# Autodesk Inventor assembly: FLUGGER R UPSTOP FLAP
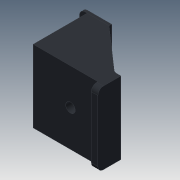
[picture p0: Inventor's stored thumbnail of the model, 180x180]
Saved by Autodesk Inventor 2020.3 (Build 243373000, 373)
## iProperties
RuleStatus: InUse
AfterDocSave0: file://Part Number Cleaner
Created: 2023-03-27
Catalog Web Link: https://www.janelia.org/
Vendor: HHMI: JRC - jET
Document SubType Name: Assembly
Designer: arnoldj
DESIGN DEPARTMENT: HHMI: JRC - jET
ALTERED ITEM PART NUMBER: N/A
ALTERED ITEM VENDOR: N/A
ALTERED ITEM DESCRIPTION: N/A
PART NUMBER - LEGACY: Standard
Author: arnoldj
Revision Number: 0
## Documents named in this file (5)
- C:\_WORKSPACE\DATA\PROJECTS\_PROJECTS BY LAB\CARD (LAB)\FLUGGER\FLUGGER R UPSTOP FLAP.iam
- C:\_WORKSPACE\DATA\PROJECTS\_PROJECTS BY LAB\CARD (LAB)\FLUGGER\FLUGGER TRAY UPSTOP FLAP .ipt
- C:\_WORKSPACE\DATA\COMMON\McMaster\94855A279_LOW-STRENGTH STEEL SQUARE NUT.ipt
- C:\_WORKSPACE\DATA\PROJECTS\_PROJECTS BY LAB\CARD (LAB)\FLUGGER\FL UPSTOP FLAP.ipt
- C:\_WORKSPACE\DATA\COMMON\McMaster\MCMASTER 91771A080 2-56 x437L FHMS SS.ipt
## Components (8 placed, 4 different names)
1. FLUGGER TRAY UPSTOP FLAP :1 — Mate:1, Mate:2, Mate:3, Mate:4, Mate:5, Mate:6, Mate:7, Mate:8, Mate:9
2. 94855A279_LOW-STRENGTH STEEL SQUARE NUT:1 — Mate:1, Mate:4
3. 94855A279_LOW-STRENGTH STEEL SQUARE NUT:2 — Mate:2, Mate:5
4. 94855A279_LOW-STRENGTH STEEL SQUARE NUT:3 — Mate:3, Mate:6
5. FL UPSTOP FLAP:1 — Mate:7, Mate:8, Mate:9, Flush:1, Mate:10, Flush:2, Mate:11, Flush:3, Mate:12
6. MCMASTER 91771A080 2-56 x437L FHMS SS:1 — Flush:3, Mate:12
7. MCMASTER 91771A080 2-56 x437L FHMS SS:2 — Flush:2, Mate:11
8. MCMASTER 91771A080 2-56 x437L FHMS SS:3 — Flush:1, Mate:10
## Relationships (15: Mate 12, Flush 3)
- Mate:1: FLUGGER TRAY UPSTOP FLAP :1 ↔ 94855A279_LOW-STRENGTH STEEL SQUARE NUT:1
- Mate:2: FLUGGER TRAY UPSTOP FLAP :1 ↔ 94855A279_LOW-STRENGTH STEEL SQUARE NUT:2
- Mate:3: FLUGGER TRAY UPSTOP FLAP :1 ↔ 94855A279_LOW-STRENGTH STEEL SQUARE NUT:3
- Mate:4: FLUGGER TRAY UPSTOP FLAP :1 ↔ 94855A279_LOW-STRENGTH STEEL SQUARE NUT:1
- Mate:5: FLUGGER TRAY UPSTOP FLAP :1 ↔ 94855A279_LOW-STRENGTH STEEL SQUARE NUT:2
- Mate:6: FLUGGER TRAY UPSTOP FLAP :1 ↔ 94855A279_LOW-STRENGTH STEEL SQUARE NUT:3
- Mate:7: FLUGGER TRAY UPSTOP FLAP :1 ↔ FL UPSTOP FLAP:1
- Mate:8: FLUGGER TRAY UPSTOP FLAP :1 ↔ FL UPSTOP FLAP:1
- Mate:9: FLUGGER TRAY UPSTOP FLAP :1 ↔ FL UPSTOP FLAP:1
- Flush:1: FL UPSTOP FLAP:1 ↔ MCMASTER 91771A080 2-56 x437L FHMS SS:3
- Mate:10: FL UPSTOP FLAP:1 ↔ MCMASTER 91771A080 2-56 x437L FHMS SS:3
- Flush:2: FL UPSTOP FLAP:1 ↔ MCMASTER 91771A080 2-56 x437L FHMS SS:2
- Mate:11: FL UPSTOP FLAP:1 ↔ MCMASTER 91771A080 2-56 x437L FHMS SS:2
- Flush:3: FL UPSTOP FLAP:1 ↔ MCMASTER 91771A080 2-56 x437L FHMS SS:1
- Mate:12: FL UPSTOP FLAP:1 ↔ MCMASTER 91771A080 2-56 x437L FHMS SS:1
